# Autodesk Inventor assembly: 装配体
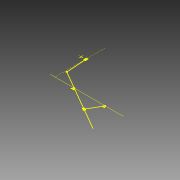
[picture p0: Inventor's stored thumbnail of the model, 180x180]
Saved by Autodesk Inventor 2013 (Build 170138000, 138)
## iProperties
Created: 2012-04-28
Part Number: 装配体
Document SubType Name: Assembly
Designer: Zhensheng
Author: Zhensheng
## Documents named in this file (8)
- E:\inventor\插床概念草图\装配体.iam
- E:\inventor\插床概念草图\草图.ipt
- E:\inventor\插床概念草图\机架one.iam
- E:\inventor\插床概念草图\滑块.ipt
- E:\inventor\插床概念草图\曲柄.ipt
- E:\inventor\插床概念草图\摇杆.ipt
- E:\inventor\插床概念草图\连杆.ipt
- E:\inventor\插床概念草图\导路.ipt
## Components (8 placed, 7 different names)
1. 草图:1
2. 机架one:1 [sub-assembly] — 配合:5, 配合:6
3. 滑块:1 — 配合:1, 配合:3
4. 曲柄:1 — 配合:3, 配合:6, 角度:1
5. 摇杆:1 — 配合:1, 配合:2, 配合:5
6. 连杆:1 — 配合:2, 配合:4
7. 滑块:2 — 表面齐平:1, 配合:4
8. 导路:1 — 表面齐平:1
## Relationships (15: Composite 7, Mate 6, Flush 1, Angle 1)
- [Composite]: 草图:1 ↔ 机架one:1
- [Composite]: 草图:1 ↔ 滑块:1
- [Composite]: 草图:1 ↔ 曲柄:1
- [Composite]: 草图:1 ↔ 摇杆:1
- [Composite]: 草图:1 ↔ 连杆:1
- [Composite]: 草图:1 ↔ 滑块:2
- [Composite]: 草图:1 ↔ 导路:1
- 配合:1 [Mate]: 滑块:1 ↔ 摇杆:1
- 配合:2 [Mate]: 摇杆:1 ↔ 连杆:1
- 表面齐平:1 [Flush]: 滑块:2 ↔ 导路:1
- 配合:3 [Mate]: 滑块:1 ↔ 曲柄:1
- 配合:4 [Mate]: 连杆:1 ↔ 滑块:2
- 配合:5 [Mate]: 机架one:1 ↔ 摇杆:1
- 配合:6 [Mate]: 机架one:1 ↔ 曲柄:1
- 角度:1 [Angle] (-120 deg): 曲柄:1
